# Autodesk Inventor assembly: STAGE1,ELEVATOR
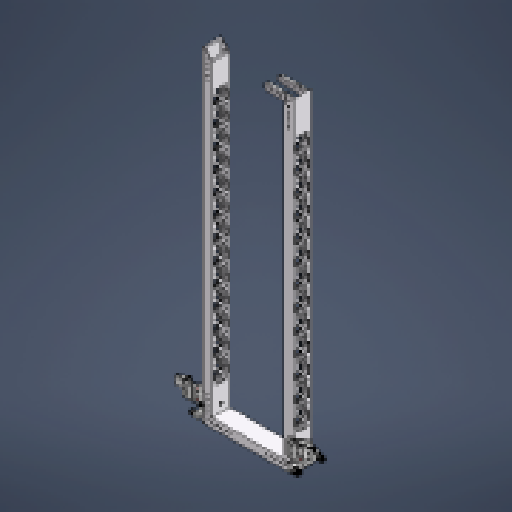
[picture p0: Inventor's stored thumbnail of the model, 512x512]
Saved by Autodesk Inventor 2024.3 (Build 283343000, 343)
## iProperties
ILogicPurgeVersion: 0.0.0.0
OnSaveVersion: 3.5.0.0
OnSaveAssembly: COREAutomationManager
Created: 2025-02-04
Part Number: STAGE1,ELEVATOR
Document SubType Name: Assembly
Designer: Jthib
Mfg Approved By: John.Thibert
Mass: 2890.66 g
Surface Area: 6308.95 cm^2
Volume: 985.653 cm^3
Density: 2.93273 g/cm^3
ModelCat: Uncategorized
CN_MASS: 2.89
Author: Jthib
## Documents named in this file (13)
- \\clfs\homes\john.thibert\2025-Poseidon-Mechanical\STAGE1,ELEVATOR.iam
- \\clfs\homes\john.thibert\2025-Poseidon-Mechanical\TUBE,ELEVATOR,SIDE,STAGE1.ipt
- \\clfs\homes\john.thibert\2025-Poseidon-Mechanical\TUBE,ELEVATOR,BOT,STAGE1.ipt
- \\clfs\homes\john.thibert\2025-Poseidon-Mechanical\PLATE,BRACKET,ELEVATOR,STAGE1.ipt
- \\clfs\homes\john.thibert\2025-Poseidon-Mechanical\SLIDE,ELEVATOR,STAGE1,LH.iam
- \\clfs\homes\john.thibert\2025-Poseidon-Mechanical\SLIDE,ELEVATOR,STAGE1,RH.iam
- \\clfs\homes\john.thibert\2025-Poseidon-Mechanical\BRACE,CHAIN,#25,ELEVATOR.ipt
- \\clfs\homes\john.thibert\2025-Poseidon-Mechanical\60355K336_Ball Bearing.ipt
- \\clfs\homes\john.thibert\2025-Poseidon-Mechanical\91259A171_Alloy Steel Shoulder Screw.ipt
- \\clfs\homes\john.thibert\2025-Poseidon-Mechanical\BEARING,MOUNT,SIDE,ELEVATOR,MIRR.ipt
- \\clfs\homes\john.thibert\2025-Poseidon-Mechanical\BEARING,MOUNT,SIDE,ELEVATOR.ipt
- \\clfs\homes\john.thibert\2025-Poseidon-Mechanical\BLOCK,BEARING,ARM,ELEVATOR.ipt
- \\clfs\homes\john.thibert\2025-Poseidon-Mechanical\TOP,BEARING_BLOCK,ELEVATOR.ipt
## Components (21 placed, 14 different names)
1. SLIDE,ELEVATOR,STAGE1,LH.iam:1 [sub-assembly] — Mate:15, Mate:16, Mate:17, Mate:18
2. SLIDE,ELEVATOR,STAGE1,RH.iam:1 [sub-assembly] — Mate:46
3. TUBE,ELEVATOR,BOT,STAGE1.ipt:1 — Mate:14, Mate:19, Mate:20, Mate:22, Mate:23, Mate:41, Mate:42
4. TUBE,ELEVATOR,SIDE,STAGE1.ipt:1 — Mate:13, Mate:48, Mate:49, Mate:50, Mate:51, Mate:52, Mate:53, Mate:54
5. TUBE,ELEVATOR,SIDE,STAGE1.ipt:2 — Mate:43, Mate:44, Mate:45, Mate:46, Mate:47, Mate:55, Mate:56, Mate:57
6. BRACE,CHAIN,#25,ELEVATOR.ipt:1
7. PLATE,BRACKET,ELEVATOR,STAGE1.ipt:2 — Mate:42, Mate:44
8. PLATE,BRACKET,ELEVATOR,STAGE1.ipt:1
9. BRACE,CHAIN,#25,ELEVATOR:2 — Mate:16, Mate:17, Mate:18
10. PLATE,BRACKET,ELEVATOR,STAGE1:4 — Mate:19, Mate:20, Mate:48, Mate:49, Mate:50
11. PLATE,BRACKET,ELEVATOR,STAGE1:5 — Mate:22, Mate:23, Mate:41, Mate:43, Mate:45, Mate:47
12. BEARING,MOUNT,SIDE,ELEVATOR:1
13. 91259A171_Alloy Steel Shoulder Screw:2
14. 60355K336_Ball Bearing:2
15. BEARING,MOUNT,SIDE,ELEVATOR,MIRR:1
16. 60355K336_Ball Bearing:1
17. 91259A171_Alloy Steel Shoulder Screw:1
18. BLOCK,BEARING,ARM,ELEVATOR:1 — Mate:51, Mate:52, Mate:53, Mate:54, Mate:58, Mate:59
19. BLOCK,BEARING,ARM,ELEVATOR:3 — Mate:55, Mate:56, Mate:57, Mate:60, Mate:61
20. TOP,BEARING_BLOCK,ELEVATOR:1 — Mate:58, Mate:59
21. TOP,BEARING_BLOCK,ELEVATOR:2 — Mate:60, Mate:61
## Relationships (54: Mate 48, Insert 6)
- [Insert]: TUBE,ELEVATOR,BOT,STAGE1.ipt:1 ↔ PLATE,BRACKET,ELEVATOR,STAGE1.ipt:1
- [Insert]: TUBE,ELEVATOR,BOT,STAGE1.ipt:1 ↔ PLATE,BRACKET,ELEVATOR,STAGE1.ipt:1
- [Insert]: TUBE,ELEVATOR,BOT,STAGE1.ipt:1 ↔ PLATE,BRACKET,ELEVATOR,STAGE1.ipt:2
- [Insert]: TUBE,ELEVATOR,BOT,STAGE1.ipt:1 ↔ PLATE,BRACKET,ELEVATOR,STAGE1.ipt:2
- [Mate]: SLIDE,ELEVATOR,STAGE1,RH.iam:1 ↔ TUBE,ELEVATOR,SIDE,STAGE1.ipt:2
- [Mate]: SLIDE,ELEVATOR,STAGE1,RH.iam:1 ↔ TUBE,ELEVATOR,SIDE,STAGE1.ipt:2
- [Mate]: SLIDE,ELEVATOR,STAGE1,LH.iam:1 ↔ TUBE,ELEVATOR,SIDE,STAGE1.ipt:1
- [Mate]: SLIDE,ELEVATOR,STAGE1,LH.iam:1 ↔ TUBE,ELEVATOR,SIDE,STAGE1.ipt:1
- [Mate]: SLIDE,ELEVATOR,STAGE1,RH.iam:1 ↔ BRACE,CHAIN,#25,ELEVATOR.ipt:1
- [Mate]: SLIDE,ELEVATOR,STAGE1,RH.iam:1 ↔ BRACE,CHAIN,#25,ELEVATOR.ipt:1
- [Mate]: SLIDE,ELEVATOR,STAGE1,RH.iam:1 ↔ BRACE,CHAIN,#25,ELEVATOR.ipt:1
- Mate:13 (-127 mm): TUBE,ELEVATOR,SIDE,STAGE1.ipt:1
- Mate:14 (-457.2 mm): TUBE,ELEVATOR,BOT,STAGE1.ipt:1
- Mate:15: SLIDE,ELEVATOR,STAGE1,LH.iam:1
- Mate:16: SLIDE,ELEVATOR,STAGE1,LH.iam:1 ↔ BRACE,CHAIN,#25,ELEVATOR:2
- Mate:17: SLIDE,ELEVATOR,STAGE1,LH.iam:1 ↔ BRACE,CHAIN,#25,ELEVATOR:2
- Mate:18: SLIDE,ELEVATOR,STAGE1,LH.iam:1 ↔ BRACE,CHAIN,#25,ELEVATOR:2
- Mate:19: TUBE,ELEVATOR,BOT,STAGE1.ipt:1 ↔ PLATE,BRACKET,ELEVATOR,STAGE1:4
- Mate:20: TUBE,ELEVATOR,BOT,STAGE1.ipt:1 ↔ PLATE,BRACKET,ELEVATOR,STAGE1:4
- Mate:22: TUBE,ELEVATOR,BOT,STAGE1.ipt:1 ↔ PLATE,BRACKET,ELEVATOR,STAGE1:5
- Mate:23: TUBE,ELEVATOR,BOT,STAGE1.ipt:1 ↔ PLATE,BRACKET,ELEVATOR,STAGE1:5
- [Mate]: 60355K336_Ball Bearing:1 ↔ 91259A171_Alloy Steel Shoulder Screw:1
- [Mate]: BRACE,CHAIN,#25,ELEVATOR.ipt:1 ↔ BEARING,MOUNT,SIDE,ELEVATOR,MIRR:1
- [Mate]: BRACE,CHAIN,#25,ELEVATOR.ipt:1 ↔ BEARING,MOUNT,SIDE,ELEVATOR,MIRR:1
- [Mate]: BRACE,CHAIN,#25,ELEVATOR.ipt:1 ↔ BEARING,MOUNT,SIDE,ELEVATOR,MIRR:1
- [Insert]: BEARING,MOUNT,SIDE,ELEVATOR,MIRR:1 ↔ 60355K336_Ball Bearing:1
- [Mate]: 60355K336_Ball Bearing:1 ↔ 91259A171_Alloy Steel Shoulder Screw:1
- [Mate]: 91259A171_Alloy Steel Shoulder Screw:2 ↔ 60355K336_Ball Bearing:2
- [Mate]: 91259A171_Alloy Steel Shoulder Screw:2 ↔ 60355K336_Ball Bearing:2
- [Insert]: BEARING,MOUNT,SIDE,ELEVATOR:1 ↔ 91259A171_Alloy Steel Shoulder Screw:2
- [Mate]: BRACE,CHAIN,#25,ELEVATOR:2 ↔ BEARING,MOUNT,SIDE,ELEVATOR:1
- [Mate]: BRACE,CHAIN,#25,ELEVATOR:2 ↔ BEARING,MOUNT,SIDE,ELEVATOR:1
- [Mate]: BRACE,CHAIN,#25,ELEVATOR:2 ↔ BEARING,MOUNT,SIDE,ELEVATOR:1
- Mate:41: TUBE,ELEVATOR,BOT,STAGE1.ipt:1 ↔ PLATE,BRACKET,ELEVATOR,STAGE1:5
- Mate:42: TUBE,ELEVATOR,BOT,STAGE1.ipt:1 ↔ PLATE,BRACKET,ELEVATOR,STAGE1.ipt:2
- Mate:43: TUBE,ELEVATOR,SIDE,STAGE1.ipt:2 ↔ PLATE,BRACKET,ELEVATOR,STAGE1:5
- Mate:44: TUBE,ELEVATOR,SIDE,STAGE1.ipt:2 ↔ PLATE,BRACKET,ELEVATOR,STAGE1.ipt:2
- Mate:45: TUBE,ELEVATOR,SIDE,STAGE1.ipt:2 ↔ PLATE,BRACKET,ELEVATOR,STAGE1:5
- Mate:46: SLIDE,ELEVATOR,STAGE1,RH.iam:1 ↔ TUBE,ELEVATOR,SIDE,STAGE1.ipt:2
- Mate:47: TUBE,ELEVATOR,SIDE,STAGE1.ipt:2 ↔ PLATE,BRACKET,ELEVATOR,STAGE1:5
- Mate:48: TUBE,ELEVATOR,SIDE,STAGE1.ipt:1 ↔ PLATE,BRACKET,ELEVATOR,STAGE1:4
- Mate:49: TUBE,ELEVATOR,SIDE,STAGE1.ipt:1 ↔ PLATE,BRACKET,ELEVATOR,STAGE1:4
- Mate:50: TUBE,ELEVATOR,SIDE,STAGE1.ipt:1 ↔ PLATE,BRACKET,ELEVATOR,STAGE1:4
- Mate:51: TUBE,ELEVATOR,SIDE,STAGE1.ipt:1 ↔ BLOCK,BEARING,ARM,ELEVATOR:1
- Mate:52: TUBE,ELEVATOR,SIDE,STAGE1.ipt:1 ↔ BLOCK,BEARING,ARM,ELEVATOR:1
- Mate:53: TUBE,ELEVATOR,SIDE,STAGE1.ipt:1 ↔ BLOCK,BEARING,ARM,ELEVATOR:1
- Mate:54: TUBE,ELEVATOR,SIDE,STAGE1.ipt:1 ↔ BLOCK,BEARING,ARM,ELEVATOR:1
- Mate:55: TUBE,ELEVATOR,SIDE,STAGE1.ipt:2 ↔ BLOCK,BEARING,ARM,ELEVATOR:3
- Mate:56: TUBE,ELEVATOR,SIDE,STAGE1.ipt:2 ↔ BLOCK,BEARING,ARM,ELEVATOR:3
- Mate:57: TUBE,ELEVATOR,SIDE,STAGE1.ipt:2 ↔ BLOCK,BEARING,ARM,ELEVATOR:3
- Mate:58: BLOCK,BEARING,ARM,ELEVATOR:1 ↔ TOP,BEARING_BLOCK,ELEVATOR:1
- Mate:59: BLOCK,BEARING,ARM,ELEVATOR:1 ↔ TOP,BEARING_BLOCK,ELEVATOR:1
- Mate:60: BLOCK,BEARING,ARM,ELEVATOR:3 ↔ TOP,BEARING_BLOCK,ELEVATOR:2
- Mate:61: BLOCK,BEARING,ARM,ELEVATOR:3 ↔ TOP,BEARING_BLOCK,ELEVATOR:2
## Named parameters: d1097_d52 = 0 mm, d1156_d1097_d52 = 0 mm, d1158_d1102 = 0 mm
